# Autodesk Inventor assembly: GearBox and Mec
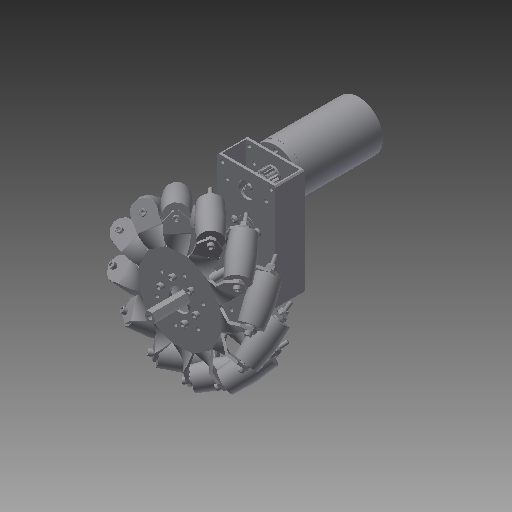
[picture p0: Inventor's stored thumbnail of the model, 512x512]
Saved by Autodesk Inventor 2018 (Build 220112000, 112)
## iProperties
Created: 2016-01-10
Part Number: GearBox and Mec
Document SubType Name: Assembly
Designer: Applefamily
Author: Applefamily
## Documents named in this file (3)
- C:\Users\Apple\Documents\Inventor\2018 PowerUp\2016_Files_2018_Mod\Assembly\GearBox and Mec.iam
- C:\Users\Apple\Documents\Inventor\2018 PowerUp\2016_Files_2018_Mod\Assembly\Imported Components\Toughbox+Nano+All+Shafts+v2\Toughbox+Nano+All+Shafts+v2.iam
- C:\Users\Apple\Documents\Inventor\2018 PowerUp\2016_Files_2018_Mod\Assembly\Imported Components\8-mecanum-right-with-roller\8-mecanum-right-with-roller.iam
## Components (2 placed, 2 different names)
1. Toughbox+Nano+All+Shafts+v2:1 [sub-assembly] — Cylindrical:1
2. 8-mecanum-right-with-roller:1 [sub-assembly] — Cylindrical:1
## Relationships (1: CylindricalJoint 1)
- Cylindrical:1: Toughbox+Nano+All+Shafts+v2:1 ↔ 8-mecanum-right-with-roller:1
